# Autodesk Inventor assembly: intake_base
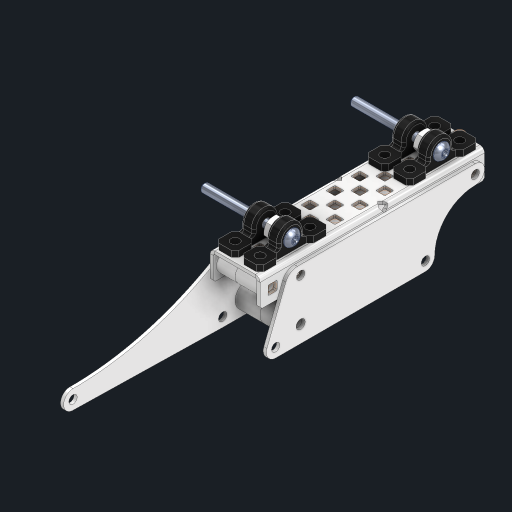
[picture p0: Inventor's stored thumbnail of the model, 512x512]
Saved by Autodesk Inventor 2024 (Build 280153000, 153)
## iProperties
Created: 2023-08-21
Part Number: intake_base
Document SubType Name: Assembly
Designer: Averey
Author: Averey
## Documents named in this file (14)
- D:\vex_robotics\hardware\cad\scrap_v0.1\intake\intake_base.iam
- D:\vex_robotics\hardware\cad\VEX-CAD-Inventor-1.41\Motion\Shaft LS\LS Pillow Bearing Block.ipt
- D:\vex_robotics\hardware\cad\VEX-CAD-Inventor-1.41\Structure\C Channel\Aluminum 1x2x1\Alu C 1x2x1x9.ipt
- D:\vex_robotics\hardware\cad\scrap_v0.1\intake\custom_parts\intake_base.ipt
- D:\vex_robotics\hardware\cad\scrap_v0.1\intake\custom_parts\intake_base_outer.ipt
- D:\vex_robotics\hardware\cad\VEX-CAD-Inventor-1.41\Motion\Spacers\Spacer Nylon .500 OD\NSpacer White .500 OD x .500.ipt
- C:\Users\Averey\Documents\vex\cad\VEX-CAD-Inventor-1.41\Motion\Spacers\Spacer Nylon .500 OD.ipt
- D:\vex_robotics\hardware\cad\VEX-CAD-Inventor-1.41\Structure\Hardware\Nut Nylon\Nut Nylon - White.ipt
- C:\Users\Averey\Documents\vex\cad\VEX-CAD-Inventor-1.41\Structure\Hardware\Nut Nylon.ipt
- D:\vex_robotics\hardware\cad\VEX-CAD-Inventor-1.41\Structure\Hardware\Screw Steel - Star\SScrew Star Smooth 1.750.ipt
- C:\Users\Averey\Documents\vex\cad\VEX-CAD-Inventor-1.41\Structure\Hardware\Screw Steel - Star.ipt
- D:\vex_robotics\hardware\cad\VEX-CAD-Inventor-1.41\Motion\Spacers\Spacer Nylon .313 OD\NSpacer .313 OD x .375.ipt
- C:\Users\Averey\Documents\vex\cad\VEX-CAD-Inventor-1.41\Motion\Spacers\Spacer Nylon .313 OD.ipt
- D:\vex_robotics\hardware\cad\VEX-CAD-Inventor-1.41\Motion\Spacers\Spacer Nylon .313 OD\NSpacer .313 OD x .500.ipt
## Components (17 placed, 9 different names)
1. intake_base:1 — Insert:8
2. intake_base_outer:1 — Insert:17, Mate:7
3. Alu C 1x2x1x9:1 — Insert:3, Mate:3, Insert:4, Mate:4, Insert:5, Insert:6, Mate:5, Mate:6, Insert:14, Insert:16, Insert:17, Mate:7
4. LS Pillow Bearing Block:1 — Insert:3, Mate:3
5. LS Pillow Bearing Block:2 — Insert:4, Mate:4, Insert:9, Insert:10
6. LS Pillow Bearing Block:3 — Insert:5, Mate:5
7. LS Pillow Bearing Block:4 — Insert:6, Mate:6, Insert:11, Insert:12
8. NSpacer White .500 OD x .500:1 — Insert:7
9. NSpacer White .500 OD x .500:2 — Insert:7, Insert:8
10. Nut Nylon - White:1 — Insert:9
11. SScrew Star Smooth 1.750:1 — Insert:10
12. Nut Nylon - White:2 — Insert:11
13. SScrew Star Smooth 1.750:2 — Insert:12
14. NSpacer .313 OD x .375:1 — Insert:13, Insert:14
15. NSpacer .313 OD x .500:2 — Insert:13
16. NSpacer .313 OD x .375:3
17. NSpacer .313 OD x .500:4 — Insert:16
## Relationships (20: Insert 15, Mate 5)
- Insert:3: Alu C 1x2x1x9:1 ↔ LS Pillow Bearing Block:1
- Mate:3: Alu C 1x2x1x9:1 ↔ LS Pillow Bearing Block:1
- Insert:4: Alu C 1x2x1x9:1 ↔ LS Pillow Bearing Block:2
- Mate:4: Alu C 1x2x1x9:1 ↔ LS Pillow Bearing Block:2
- Insert:5: Alu C 1x2x1x9:1 ↔ LS Pillow Bearing Block:3
- Insert:6: Alu C 1x2x1x9:1 ↔ LS Pillow Bearing Block:4
- Mate:5: Alu C 1x2x1x9:1 ↔ LS Pillow Bearing Block:3
- Mate:6: Alu C 1x2x1x9:1 ↔ LS Pillow Bearing Block:4
- Insert:7: NSpacer White .500 OD x .500:1 ↔ NSpacer White .500 OD x .500:2
- Insert:8: intake_base:1 ↔ NSpacer White .500 OD x .500:2
- Insert:9: LS Pillow Bearing Block:2 ↔ Nut Nylon - White:1
- Insert:10: LS Pillow Bearing Block:2 ↔ SScrew Star Smooth 1.750:1
- Insert:11: LS Pillow Bearing Block:4 ↔ Nut Nylon - White:2
- Insert:12: LS Pillow Bearing Block:4 ↔ SScrew Star Smooth 1.750:2
- Insert:13: NSpacer .313 OD x .375:1 ↔ NSpacer .313 OD x .500:2
- Insert:14: Alu C 1x2x1x9:1 ↔ NSpacer .313 OD x .375:1
- [Insert]: NSpacer .313 OD x .375:3 ↔ NSpacer .313 OD x .500:4
- Insert:16: Alu C 1x2x1x9:1 ↔ NSpacer .313 OD x .500:4
- Insert:17: intake_base_outer:1 ↔ Alu C 1x2x1x9:1
- Mate:7: intake_base_outer:1 ↔ Alu C 1x2x1x9:1
## Named parameters: d107_d105 = 0 mm
